# Autodesk Inventor assembly: Assembly1
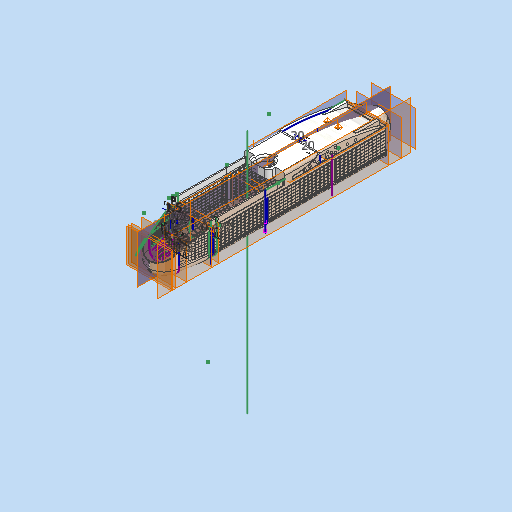
[picture p0: Inventor's stored thumbnail of the model, 512x512]
Saved by Autodesk Inventor 2027 (Build 310192060, 192F)
## iProperties
Created: 2026-08-07
Part Number: Assembly1
Document SubType Name: Assembly
Designer: mateo
Author: mateo
## Documents named in this file (3)
- C:\GitHub\SWIFT-UAV\System_development\Pelican\structural_model\v0.3.0\Parts\STEP\Assembly1.iam
- C:\GitHub\SWIFT-UAV\System_development\Pelican\structural_model\v0.3.1\Parts\Wings\WingBox.ipt
- C:\GitHub\SWIFT-UAV\System_development\Pelican\structural_model\v0.3.1\Parts\Fuselage\FuselageV2.ipt
## Components (2 placed, 2 different names)
1. WingBox:1 — Mate:1
2. FuselageV2:1 — Mate:1
## Relationships (1: Mate 1)
- Mate:1: WingBox:1 ↔ FuselageV2:1
